# Autodesk Inventor assembly: wheelForHangingAndMovingV2
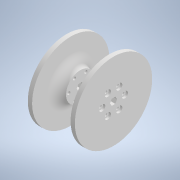
[picture p0: Inventor's stored thumbnail of the model, 180x180]
Saved by Autodesk Inventor 2020.2 (Build 242310000, 310)
## iProperties
Created: 2020-01-09
Part Number: wheelForHangingAndMovingV2
Document SubType Name: Assembly
Designer: robst
Author: robst
## Documents named in this file (2)
- C:\git\CAD-Development\robSteele\2020 Lift Mechanism\wheelForHangingAndMovingV2.iam
- C:\git\CAD-Development\robSteele\2020 Lift Mechanism\halfWheelForHangingAndMovingV2.ipt
## Components (2 placed, 1 different names)
1. halfWheelForHangingAndMovingV2:1 — Mate:1, Mate:2
2. halfWheelForHangingAndMovingV2:2 — Mate:1, Mate:2
## Relationships (2: Mate 2)
- Mate:1: halfWheelForHangingAndMovingV2:1 ↔ halfWheelForHangingAndMovingV2:2
- Mate:2: halfWheelForHangingAndMovingV2:1 ↔ halfWheelForHangingAndMovingV2:2
